# Autodesk Inventor assembly: SteelStairs
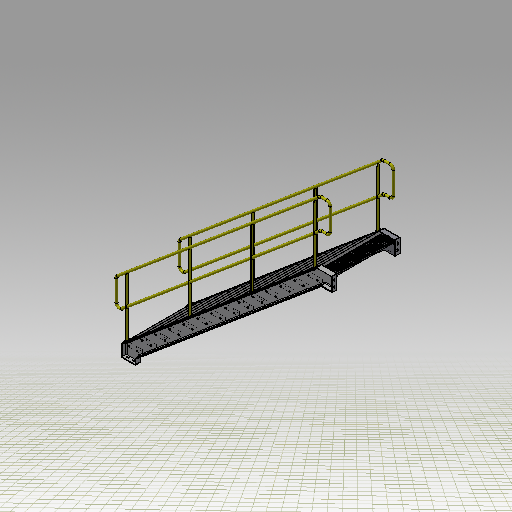
[picture p0: Inventor's stored thumbnail of the model, 512x512]
Saved by Autodesk Inventor 2026.2 (Build 302298000, 298)
## iProperties
RuleStatus: InUse
Created: 2015-03-25
Part Number: SteelStairs
Document SubType Name: Assembly
Designer: m_crauwels
Mass: 402297 g
Surface Area: 216114 cm^2
Volume: 51249.7 cm^3
Density: 7.84974 g/cm^3
m10: 800.000 mm
STAIRS_HEIGHT: 3000.000 mm
STAIRS_ANGLE: 40.00 deg
STAIRS_WIDTH: 1000.000 mm
Author: m_crauwels
## iProperties of the stored document MemberDocs/xAaaaqycaAaaaaaaaAaaaaps2Gg
RuleStatus: InUse
Created: 2015-03-25
Part Number: SteelStairs
Document SubType Name: Assembly
Designer: m_crauwels
Mass: 402297 g
Surface Area: 216114 cm^2
Volume: 51249.7 cm^3
Density: 7.84974 g/cm^3
m10: 800.000 mm
STAIRS_HEIGHT: 2200,000 mm
STAIRS_ANGLE: 37,00 deg
STAIRS_WIDTH: 1000,000 mm
Author: m_crauwels
## Documents named in this file (9)
- D:\Inventor Projects\Steel and Stairs\Stairs\Stairs.iam
- D:\Inventor Projects\Steel and Stairs\Stairs\StairsConnectionPlate.ipt
- D:\Inventor Projects\Steel and Stairs\Stairs\StairsLeftSideUPN.ipt
- D:\Inventor Projects\Steel and Stairs\Stairs\Tread.ipt
- D:\Inventor Projects\Steel and Stairs\Stairs\Railing.ipt
- D:\Inventor Projects\Steel and Stairs\Stairs\StairsRightSideUPN.ipt
- C:\Users\marc_\Documents\Inventor\Content Center Files\R2026\en-US\ISO 7089\ISO 7089 - 12 - 140 HV(1).ipt
- C:\Users\marc_\Documents\Inventor\Content Center Files\R2026\en-US\ISO 4032(2)\ISO 4032 - M12 - ISO.ipt
- C:\Users\marc_\Documents\Inventor\Content Center Files\R2026\en-US\ISO 4017(1)\ISO 4017 - M12 x 35 - ISO.ipt
## Components (327 placed, 12 different names)
1. Stairs Left UPN — Mate:5, Flush:6, Mate:6, Mate:11, Flush:7, Flush:8, Mate:12, Flush:9, Flush:10, Insert:1, Insert:2, Insert:5, Insert:6, Flush:11, Flush:12, Insert:19, Insert:20
2. Stairs Right UPN — Mate:14, Flush:11, Flush:12, Insert:11, Insert:12, Mate:15, Flush:13, Flush:14, Mate:16, Flush:15, Flush:16, Insert:35, Insert:36
3. Railing Left — Insert:1, Insert:2, Insert:3, Insert:4
4. Railing Right — Insert:11, Insert:12, Insert:27, Insert:28
5. Stairs Connectionplate Up Left — Mate:10, Mate:11, Flush:7, Flush:8
6. Stairs Connectionplate Lower Left — Mate:9, Mate:12, Flush:9, Flush:10
7. Stairs Connectionplate Up Right — Mate:15, Flush:13, Flush:14
8. Stairs Connectionplate Lower Leftt — Mate:16, Flush:15, Flush:16
9. Tread:2 — Mate:5, Flush:6, Mate:6, Mate:13, Mate:14
10. Tread:3
11. Tread:4
12. Tread:5
13. Tread:6
14. Tread:7
15. Tread:8
16. Tread:9
17. Tread:10
18. Tread:11
19. Tread:12
20. Tread:13
21. Tread:14
22. Tread:15
23. Tread:16
24. ISO 7089 12:3 — Insert:3, Insert:9
25. ISO 7089 12:4 — Insert:4, Insert:10
26. ISO 7089 12:5 — Insert:5
27. ISO 7089 12:6 — Insert:6
28. ISO 4032 M12:2
29. ISO 4032 M12:6
30. ISO 4017 M12 x 35:1 — Insert:9
31. ISO 4017 M12 x 35:2 — Insert:10
32. ISO 7089 12:7
33. ISO 7089 12:8
34. ISO 7089 12:9
35. ISO 7089 12:10
36. ISO 4032 M12:3
37. ISO 4032 M12:7
38. ISO 4017 M12 x 35:3
39. ISO 4017 M12 x 35:4
40. ISO 7089 12:11
41. ISO 7089 12:12
42. ISO 7089 12:13
43. ISO 7089 12:14
44. ISO 4032 M12:4
45. ISO 4032 M12:8
46. ISO 4017 M12 x 35:5
47. ISO 4017 M12 x 35:6
48. ISO 7089 12:15
49. ISO 7089 12:16
50. ISO 7089 12:17
51. ISO 7089 12:18
52. ISO 4032 M12:5
53. ISO 4032 M12:9
54. ISO 4017 M12 x 35:7
55. ISO 4017 M12 x 35:8
56. ISO 7089 12:19 — Insert:17
57. ISO 7089 12:20 — Insert:17, Insert:19
58. ISO 4032 M12:10
59. ISO 4017 M12 x 35:9
60. ISO 7089 12:21 — Insert:18, Insert:20
61. ISO 7089 12:22 — Insert:18
62. ISO 4032 M12:11
63. ISO 4017 M12 x 35:10
64. ISO 7089 12:23
65. ISO 7089 12:24
66. ISO 4032 M12:12
67. ISO 4017 M12 x 35:11
68. ISO 7089 12:25
69. ISO 7089 12:26
70. ISO 4032 M12:13
71. ISO 4017 M12 x 35:12
72. ISO 7089 12:27
73. ISO 7089 12:28
74. ISO 4032 M12:14
75. ISO 4017 M12 x 35:13
76. ISO 7089 12:29
77. ISO 7089 12:30
78. ISO 4032 M12:15
79. ISO 4017 M12 x 35:14
80. ISO 7089 12:31
81. ISO 7089 12:32
82. ISO 4032 M12:16
83. ISO 4017 M12 x 35:15
84. ISO 7089 12:33
85. ISO 7089 12:34
86. ISO 4032 M12:17
87. ISO 4017 M12 x 35:16
88. ISO 7089 12:35
89. ISO 7089 12:36
90. ISO 4032 M12:18
91. ISO 4017 M12 x 35:17
92. ISO 7089 12:37
93. ISO 7089 12:38
94. ISO 4032 M12:19
95. ISO 4017 M12 x 35:18
96. ISO 7089 12:39
97. ISO 7089 12:40
98. ISO 4032 M12:20
99. ISO 4017 M12 x 35:19
100. ISO 7089 12:41
101. ISO 7089 12:42
102. ISO 4032 M12:21
103. ISO 4017 M12 x 35:20
104. ISO 7089 12:43
105. ISO 7089 12:44
106. ISO 4032 M12:22
107. ISO 4017 M12 x 35:21
108. ISO 7089 12:45
109. ISO 7089 12:46
110. ISO 4032 M12:23
111. ISO 4017 M12 x 35:22
112. ISO 7089 12:47
113. ISO 7089 12:48
114. ISO 4032 M12:24
115. ISO 4017 M12 x 35:23
116. ISO 7089 12:49
117. ISO 7089 12:50
118. ISO 4032 M12:25
119. ISO 4017 M12 x 35:24
120. ISO 7089 12:51
121. ISO 7089 12:52
122. ISO 4032 M12:26
123. ISO 4017 M12 x 35:25
124. ISO 7089 12:53
125. ISO 7089 12:54
126. ISO 4032 M12:27
127. ISO 4017 M12 x 35:26
128. ISO 7089 12:55
129. ISO 7089 12:56
130. ISO 4032 M12:28
131. ISO 4017 M12 x 35:27
132. ISO 7089 12:57
133. ISO 7089 12:58
134. ISO 4032 M12:29
135. ISO 4017 M12 x 35:28
136. ISO 7089 12:59
137. ISO 7089 12:60
138. ISO 4032 M12:30
139. ISO 4017 M12 x 35:29
140. ISO 7089 12:61
141. ISO 7089 12:62
142. ISO 4032 M12:31
143. ISO 4017 M12 x 35:30
144. ISO 7089 12:63
145. ISO 7089 12:64
146. ISO 4032 M12:32
147. ISO 4017 M12 x 35:31
148. ISO 7089 12:65
149. ISO 7089 12:66
150. ISO 4032 M12:33
151. ISO 4017 M12 x 35:32
152. ISO 7089 12:67
153. ISO 7089 12:68
154. ISO 4032 M12:34
155. ISO 4017 M12 x 35:33
156. ISO 7089 12:69
157. ISO 7089 12:70
158. ISO 4032 M12:35
159. ISO 4017 M12 x 35:34
160. ISO 7089 12:71
161. ISO 7089 12:72
162. ISO 4032 M12:36
163. ISO 4017 M12 x 35:35
164. ISO 7089 12:73
165. ISO 7089 12:74
166. ISO 4032 M12:37
167. ISO 4017 M12 x 35:36
168. ISO 7089 12:75
169. ISO 7089 12:76
170. ISO 4032 M12:38
171. ISO 4017 M12 x 35:37
172. ISO 7089 12:77
173. ISO 7089 12:78
174. ISO 4032 M12:39
175. ISO 4017 M12 x 35:38
176. ISO 7089 12:79 — Insert:26, Insert:27
177. ISO 7089 12:80 — Insert:25, Insert:28
178. ISO 7089 12:81 — Insert:26
179. ISO 7089 12:82 — Insert:25
180. ISO 4032 M12:40
181. ISO 4032 M12:41
182. ISO 4017 M12 x 35:39
183. ISO 4017 M12 x 35:40
184. ISO 7089 12:83
185. ISO 7089 12:84
186. ISO 7089 12:85
187. ISO 7089 12:86
188. ISO 4032 M12:42
189. ISO 4032 M12:43
190. ISO 4017 M12 x 35:41
191. ISO 4017 M12 x 35:42
192. ISO 7089 12:87
193. ISO 7089 12:88
194. ISO 7089 12:89
195. ISO 7089 12:90
196. ISO 4032 M12:44
197. ISO 4032 M12:45
198. ISO 4017 M12 x 35:43
199. ISO 4017 M12 x 35:44
200. ISO 7089 12:91
201. ISO 7089 12:92
202. ISO 7089 12:93
203. ISO 7089 12:94
204. ISO 4032 M12:46
205. ISO 4032 M12:47
206. ISO 4017 M12 x 35:45
207. ISO 4017 M12 x 35:46
208. ISO 7089 12:95 — Insert:35
209. ISO 7089 12:96
210. ISO 4032 M12:48
211. ISO 4017 M12 x 35:47
212. ISO 7089 12:97 — Insert:36
213. ISO 7089 12:98
214. ISO 4032 M12:49
215. ISO 4017 M12 x 35:48
216. ISO 7089 12:99
217. ISO 7089 12:100
218. ISO 4032 M12:50
219. ISO 4017 M12 x 35:49
220. ISO 7089 12:101
221. ISO 7089 12:102
222. ISO 4032 M12:51
223. ISO 4017 M12 x 35:50
224. ISO 7089 12:103
225. ISO 7089 12:104
226. ISO 4032 M12:52
227. ISO 4017 M12 x 35:51
228. ISO 7089 12:105
229. ISO 7089 12:106
230. ISO 4032 M12:53
231. ISO 4017 M12 x 35:52
232. ISO 7089 12:107
233. ISO 7089 12:108
234. ISO 4032 M12:54
235. ISO 4017 M12 x 35:53
236. ISO 7089 12:109
237. ISO 7089 12:110
238. ISO 4032 M12:55
239. ISO 4017 M12 x 35:54
240. ISO 7089 12:111
241. ISO 7089 12:112
242. ISO 4032 M12:56
243. ISO 4017 M12 x 35:55
244. ISO 7089 12:113
245. ISO 7089 12:114
246. ISO 4032 M12:57
247. ISO 4017 M12 x 35:56
248. ISO 7089 12:115
249. ISO 7089 12:116
250. ISO 4032 M12:58
251. ISO 4017 M12 x 35:57
252. ISO 7089 12:117
253. ISO 7089 12:118
254. ISO 4032 M12:59
255. ISO 4017 M12 x 35:58
256. ISO 7089 12:119
257. ISO 7089 12:120
258. ISO 4032 M12:60
259. ISO 4017 M12 x 35:59
260. ISO 7089 12:121
261. ISO 7089 12:122
262. ISO 4032 M12:61
263. ISO 4017 M12 x 35:60
264. ISO 7089 12:123
265. ISO 7089 12:124
266. ISO 4032 M12:62
267. ISO 4017 M12 x 35:61
268. ISO 7089 12:125
269. ISO 7089 12:126
270. ISO 4032 M12:63
271. ISO 4017 M12 x 35:62
272. ISO 7089 12:127
273. ISO 7089 12:128
274. ISO 4032 M12:64
275. ISO 4017 M12 x 35:63
276. ISO 7089 12:129
277. ISO 7089 12:130
278. ISO 4032 M12:65
279. ISO 4017 M12 x 35:64
280. ISO 7089 12:131
281. ISO 7089 12:132
282. ISO 4032 M12:66
283. ISO 4017 M12 x 35:65
284. ISO 7089 12:133
285. ISO 7089 12:134
286. ISO 4032 M12:67
287. ISO 4017 M12 x 35:66
288. ISO 7089 12:135
289. ISO 7089 12:136
290. ISO 4032 M12:68
291. ISO 4017 M12 x 35:67
292. ISO 7089 12:137
293. ISO 7089 12:138
294. ISO 4032 M12:69
295. ISO 4017 M12 x 35:68
296. ISO 7089 12:139
297. ISO 7089 12:140
298. ISO 4032 M12:70
299. ISO 4017 M12 x 35:69
300. ISO 7089 12:141
301. ISO 7089 12:142
302. ISO 4032 M12:71
303. ISO 4017 M12 x 35:70
304. ISO 7089 12:143
305. ISO 7089 12:144
306. ISO 4032 M12:72
307. ISO 4017 M12 x 35:71
308. ISO 7089 12:145
309. ISO 7089 12:146
310. ISO 4032 M12:73
311. ISO 4017 M12 x 35:72
312. ISO 7089 12:147
313. ISO 7089 12:148
314. ISO 4032 M12:74
315. ISO 4017 M12 x 35:73
316. ISO 7089 12:149
317. ISO 7089 12:150
318. ISO 4032 M12:75
319. ISO 4017 M12 x 35:74
320. ISO 7089 12:151
321. ISO 7089 12:152
322. ISO 4032 M12:76
323. ISO 4017 M12 x 35:75
324. ISO 7089 12:153
325. ISO 7089 12:154
326. ISO 4032 M12:77
327. ISO 4017 M12 x 35:76
## Component patterns: Steps Pattern (15 elements), Left Railing Bolts Pattern (4 elements), Left Steps Bolts Pattern (15 elements), Right Railing Bolts Pattern (4 elements), Left Railing Bolts Pattern (15 elements)
## Relationships (57: Insert 36, Flush 11, Mate 10)
- Mate:5: Stairs Left UPN ↔ Tread:2
- Flush:6: Stairs Left UPN ↔ Tread:2
- Mate:6: Stairs Left UPN ↔ Tread:2
- Mate:9: Stairs Connectionplate Lower Left
- Mate:10: Stairs Connectionplate Up Left
- Mate:11: Stairs Left UPN ↔ Stairs Connectionplate Up Left
- Flush:7: Stairs Left UPN ↔ Stairs Connectionplate Up Left
- Flush:8: Stairs Left UPN ↔ Stairs Connectionplate Up Left
- Mate:12: Stairs Left UPN ↔ Stairs Connectionplate Lower Left
- Flush:9: Stairs Left UPN ↔ Stairs Connectionplate Lower Left
- Flush:10: Stairs Left UPN ↔ Stairs Connectionplate Lower Left
- Mate:13: Tread:2
- Insert:1: Stairs Left UPN ↔ Railing Left
- Insert:2: Stairs Left UPN ↔ Railing Left
- Insert:3: Railing Left ↔ ISO 7089 12:3
- Insert:4: Railing Left ↔ ISO 7089 12:4
- Insert:5 (-15 mm): Stairs Left UPN ↔ ISO 7089 12:5
- Insert:6 (-15 mm): Stairs Left UPN ↔ ISO 7089 12:6
- [Insert]: ISO 7089 12:5 ↔ ISO 4032 M12:2
- [Insert]: ISO 7089 12:6 ↔ ISO 4032 M12:6
- Insert:9: ISO 7089 12:3 ↔ ISO 4017 M12 x 35:1
- Insert:10: ISO 7089 12:4 ↔ ISO 4017 M12 x 35:2
- Mate:14: Stairs Right UPN ↔ Tread:2
- Flush:11: Stairs Left UPN ↔ Stairs Right UPN
- Flush:12: Stairs Left UPN ↔ Stairs Right UPN
- Insert:11: Stairs Right UPN ↔ Railing Right
- Insert:12: Stairs Right UPN ↔ Railing Right
- Mate:15: Stairs Right UPN ↔ Stairs Connectionplate Up Right
- Flush:13: Stairs Right UPN ↔ Stairs Connectionplate Up Right
- Flush:14: Stairs Right UPN ↔ Stairs Connectionplate Up Right
- Mate:16: Stairs Right UPN ↔ Stairs Connectionplate Lower Leftt
- Flush:15: Stairs Right UPN ↔ Stairs Connectionplate Lower Leftt
- Flush:16: Stairs Right UPN ↔ Stairs Connectionplate Lower Leftt
- [Insert]: ISO 7089 12:19 ↔ ISO 4032 M12:10
- [Insert]: ISO 7089 12:20 ↔ ISO 4017 M12 x 35:9
- [Insert]: ISO 7089 12:22 ↔ ISO 4032 M12:11
- [Insert]: ISO 7089 12:21 ↔ ISO 4017 M12 x 35:10
- Insert:17 (13 mm): ISO 7089 12:19 ↔ ISO 7089 12:20
- Insert:18 (13 mm): ISO 7089 12:21 ↔ ISO 7089 12:22
- Insert:19: Stairs Left UPN ↔ ISO 7089 12:20
- Insert:20: Stairs Left UPN ↔ ISO 7089 12:21
- [Insert]: ISO 7089 12:81 ↔ ISO 4032 M12:40
- [Insert]: ISO 7089 12:82 ↔ ISO 4032 M12:41
- [Insert]: ISO 7089 12:79 ↔ ISO 4017 M12 x 35:39
- [Insert]: ISO 7089 12:80 ↔ ISO 4017 M12 x 35:40
- Insert:25 (15 mm): ISO 7089 12:80 ↔ ISO 7089 12:82
- Insert:26 (15 mm): ISO 7089 12:79 ↔ ISO 7089 12:81
- Insert:27: Railing Right ↔ ISO 7089 12:79
- Insert:28: Railing Right ↔ ISO 7089 12:80
- [Insert]: ISO 7089 12:96 ↔ ISO 4032 M12:48
- [Insert]: ISO 7089 12:95 ↔ ISO 4017 M12 x 35:47
- [Insert]: ISO 7089 12:98 ↔ ISO 4032 M12:49
- [Insert]: ISO 7089 12:97 ↔ ISO 4017 M12 x 35:48
- [Insert] (13 mm): ISO 7089 12:95 ↔ ISO 7089 12:96
- [Insert] (13 mm): ISO 7089 12:97 ↔ ISO 7089 12:98
- Insert:35: Stairs Right UPN ↔ ISO 7089 12:95
- Insert:36: Stairs Right UPN ↔ ISO 7089 12:97
## Named parameters: d85_d74 = 0 mm, d86_d76 = 0 mm, d87_d74 = 0 mm, d88_d76 = 0 mm, d113_d74 = 0 mm, d114_d75 = 0 mm, d115_d76 = 0 mm, d116_d77 = 0 mm, d121_d85_d74 = 0 mm, d122_d86_d76 = 0 mm, d123_d87_d74 = 0 mm, d124_d88_d76 = 0 mm, d125_d89 = 13 mm, d126_d90 = 13 mm, STAIRS_HEIGHT = 3000 mm, STAIRS_ANGLE = 40 deg, STAIRS_WIDTH = 1000 mm
